# Autodesk Inventor assembly: V2 modular session with camera for cutout 50 deg
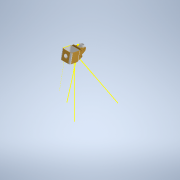
[picture p0: Inventor's stored thumbnail of the model, 180x180]
Saved by Autodesk Inventor 2020 (Build 240168000, 168)
## iProperties
Created: 2022-08-01
Part Number: V2 modular session with camera for cutout 50 deg
Document SubType Name: Assembly
Designer: Steven
Author: Steven
## Documents named in this file (3)
- Y:\FPV drone stuff\0 Street League\Frames\PB-Kauri-X\3D prints\35 mm canopy\work in progress prints\session mounts\V2 modular session with camera for cutout 50 deg.iam
- Y:\FPV drone stuff\0 Street League\Frames\PB-Kauri-X\3D prints\35 mm canopy\work in progress prints\session mounts\V2 session mount 50deg block.ipt
- Y:\FPV drone stuff\0 Street League\Frames\PB-Kauri-X\3D prints\35 mm canopy\work in progress prints\Camera mounts\predator nano\50 deg predator nano mount.ipt
## Components (2 placed, 2 different names)
1. V2 session mount 50deg block:1 — Flush:1, Flush:2, Flush:3, Flush:4, Mate:1, Mate:2
2. 50 deg predator nano mount:1 — Flush:4, Mate:1, Mate:2
## Relationships (6: Flush 4, Mate 2)
- Flush:1: V2 session mount 50deg block:1
- Flush:2: V2 session mount 50deg block:1
- Flush:3: V2 session mount 50deg block:1
- Flush:4 (6.15 mm): V2 session mount 50deg block:1 ↔ 50 deg predator nano mount:1
- Mate:1: V2 session mount 50deg block:1 ↔ 50 deg predator nano mount:1
- Mate:2: V2 session mount 50deg block:1 ↔ 50 deg predator nano mount:1
